# Autodesk Inventor assembly: draft assembly 3
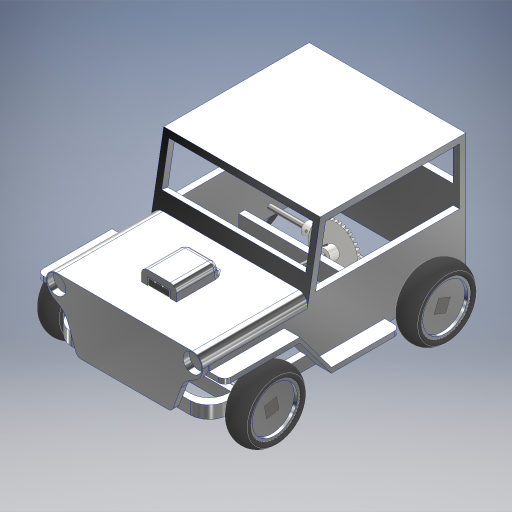
[picture p0: Inventor's stored thumbnail of the model, 512x512]
Saved by Autodesk Inventor 2024 (Build 280153000, 153)
## iProperties
Created: 2024-04-13
Part Number: draft assembly 3
Document SubType Name: Assembly
Designer: Alex
Author: Alex
## Documents named in this file (10)
- C:\Shared\alex-bartella-schoolwork\4z03\final\draft assembly 3.iam
- C:\Shared\alex-bartella-schoolwork\4z03\final\shell.ipt
- C:\Shared\alex-bartella-schoolwork\4z03\final\rc_motor\rc_motor.ipt
- C:\Shared\alex-bartella-schoolwork\4z03\final\rear axle.ipt
- C:\Shared\alex-bartella-schoolwork\4z03\final\final\wheel.iam
- C:\Shared\alex-bartella-schoolwork\4z03\final\final\gears\Bevel Gears4.iam
- C:\Users\turbo\Documents\Inventor\Content Center Files\R2024\en-US\ANSI_ASME B18.6.5M(1)\ANSI_ASME B18.6.5M - M3.5x0.6 x 20(1) T.ipt
- C:\Shared\alex-bartella-schoolwork\4z03\final\driveshaft.ipt
- C:\Shared\alex-bartella-schoolwork\4z03\final\front axle.ipt
- C:\Shared\alex-bartella-schoolwork\4z03\final\rc_battery\rc_battery.ipt
## Components (13 placed, 9 different names)
1. shell:1 — Flush:1, Flush:2, Flush:3, Mate:3, Mate:4, Mate:5, Mate:6, Mate:7, Mate:8, Mate:9, Mate:10, Mate:11, Temp:1, Temp, Mate:19, Mate:20, Mate:24, Angle:3, Mate:30, Mate:31, Mate:32
2. rc_motor:1 — Mate:15, Temp:1, Temp, Mate:17, Angle:2, Mate:18, Mate:19, Mate:20, Driver
3. rear axle:1 — Mate:11, Mate:12, Mate:13, Mate:14, Flush:5
4. wheel:1 [sub-assembly] — Mate:5, Mate:6, Mate:12
5. wheel:2 [sub-assembly] — Mate:9, Mate:10, Mate:29
6. wheel:3 [sub-assembly] — Mate:3, Mate:4, Mate:13
7. wheel:4 [sub-assembly] — Mate:7, Mate:8, Mate:27, Mate:28
8. Bevel Gears:1 [sub-assembly] — Mate:14, Mate:15, Flush:5, Mate:21, Mate:23, Mate:25, Flush:6, Mate:26, Driver
9. Slotted Flat Countersunk Head Tapping Screw - Type T - Metric M3.5x0.6 x 20:1 — Mate:21
10. driveshaft:1 — Mate:25, Flush:6, Mate:26
11. Slotted Flat Countersunk Head Tapping Screw - Type T - Metric M3.5x0.6 x 20:2 — Mate:23
12. front axle:1 — Mate:27, Mate:28, Mate:29
13. rc_battery:1 — Mate:30, Mate:31, Mate:32
## Relationships (38: Mate 28, Flush 6, Angle 4)
- Flush:1: shell:1
- Flush:2: shell:1
- Flush:3: shell:1
- Mate:3: shell:1 ↔ wheel:3
- Mate:4: shell:1 ↔ wheel:3
- Mate:5: shell:1 ↔ wheel:1
- Mate:6: shell:1 ↔ wheel:1
- Mate:7: shell:1 ↔ wheel:4
- Mate:8: shell:1 ↔ wheel:4
- Mate:9: shell:1 ↔ wheel:2
- Mate:10: shell:1 ↔ wheel:2
- Mate:11: shell:1 ↔ rear axle:1
- Mate:12: rear axle:1 ↔ wheel:1
- Mate:13: rear axle:1 ↔ wheel:3
- Mate:14: rear axle:1 ↔ Bevel Gears:1
- Mate:15: rc_motor:1 ↔ Bevel Gears:1
- Temp:1 [Angle] (84 deg): shell:1 ↔ rc_motor:1
- Temp [Flush]: shell:1 ↔ rc_motor:1
- Mate:17: rc_motor:1
- Angle:2 (0 deg): rc_motor:1
- Mate:18: rc_motor:1
- Mate:19: shell:1 ↔ rc_motor:1
- Mate:20: shell:1 ↔ rc_motor:1
- Flush:5: rear axle:1 ↔ Bevel Gears:1
- Mate:21: Bevel Gears:1 ↔ Slotted Flat Countersunk Head Tapping Screw - Type T - Metric M3.5x0.6 x 20:1
- Mate:23: Bevel Gears:1 ↔ Slotted Flat Countersunk Head Tapping Screw - Type T - Metric M3.5x0.6 x 20:2
- Mate:24: shell:1
- Angle:3 (176 deg): shell:1
- Mate:25: Bevel Gears:1 ↔ driveshaft:1
- Flush:6: Bevel Gears:1 ↔ driveshaft:1
- Mate:26: Bevel Gears:1 ↔ driveshaft:1
- Driver [Angle] (0 deg): rc_motor:1 ↔ Bevel Gears:1
- Mate:27: wheel:4 ↔ front axle:1
- Mate:28: wheel:4 ↔ front axle:1
- Mate:29: wheel:2 ↔ front axle:1
- Mate:30: shell:1 ↔ rc_battery:1
- Mate:31: shell:1 ↔ rc_battery:1
- Mate:32: shell:1 ↔ rc_battery:1
